# Autodesk Inventor assembly: Kepler Vibe Assembly
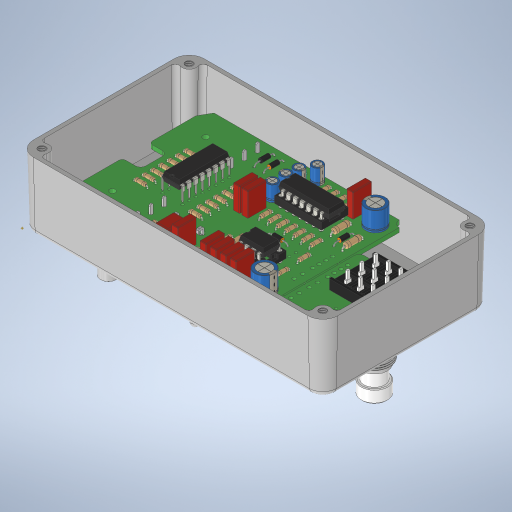
[picture p0: Inventor's stored thumbnail of the model, 512x512]
Saved by Autodesk Inventor 2023 (Build 270158030, 158C)
## iProperties
Created: 2022-11-10
Part Number: Kepler Vibe Assembly
Document SubType Name: Assembly
Designer: Imogen Heard
Author: Imogen Heard
## Documents named in this file (3)
- C:\Users\dheard\Documents\Inventor\Inventor_Projects\Electronics Projects\Kepler Vibe Assembly.iam
- C:\Users\dheard\Documents\Inventor\Inventor_Projects\Electronics Projects\Kepler Vibe Enclosure.ipt
- C:\Users\dheard\Documents\Inventor\Inventor_Projects\Electronics Projects\Kepler_Vibe_PCB_v2.ipt
## Components (2 placed, 2 different names)
1. Kepler Vibe Enclosure:1 — Mate:1, Mate:2, Mate:3
2. Kepler_Vibe_PCB_v2:1 — Mate:1, Mate:2, Mate:3
## Relationships (3: Mate 3)
- Mate:1: Kepler Vibe Enclosure:1 ↔ Kepler_Vibe_PCB_v2:1
- Mate:2 (2 mm): Kepler Vibe Enclosure:1 ↔ Kepler_Vibe_PCB_v2:1
- Mate:3 (30 mm): Kepler Vibe Enclosure:1 ↔ Kepler_Vibe_PCB_v2:1
